# Autodesk Inventor assembly: BumperBrackets
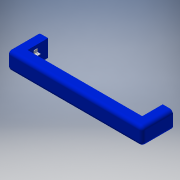
[picture p0: Inventor's stored thumbnail of the model, 180x180]
Saved by Autodesk Inventor 2016 (Build 200138000, 138)
## iProperties
Created: 2017-01-27
Part Number: BumperBrackets
Document SubType Name: Assembly
Designer: hamblettk
Author: hamblettk
## Documents named in this file (3)
- E:\1073CAD\Robot2017\DriveTrain\BumperBrackets.iam
- E:\1073CAD\Robot2017\DriveTrain\Bumper.ipt
- E:\1073CAD\Robot2017\DriveTrain\Lbracket.ipt
## Components (4 placed, 2 different names)
1. Bumper:1 — Mate:1, Mate:2, Mate:3, Mate:4, Mate:5, Flush:1, Flush:2, Mate:6, Flush:3
2. Lbracket:1 — Mate:1, Mate:5, Flush:1
3. Lbracket:2 — Mate:2, Mate:6, Flush:3
4. Lbracket:3 — Mate:3, Mate:4, Flush:2
## Relationships (9: Mate 6, Flush 3)
- Mate:1: Bumper:1 ↔ Lbracket:1
- Mate:2: Bumper:1 ↔ Lbracket:2
- Mate:3: Bumper:1 ↔ Lbracket:3
- Mate:4 (46.0375 mm): Bumper:1 ↔ Lbracket:3
- Mate:5 (46.0375 mm): Bumper:1 ↔ Lbracket:1
- Flush:1 (25.4 mm): Bumper:1 ↔ Lbracket:1
- Flush:2 (25.4 mm): Bumper:1 ↔ Lbracket:3
- Mate:6 (412.75 mm): Bumper:1 ↔ Lbracket:2
- Flush:3 (25.4 mm): Bumper:1 ↔ Lbracket:2
